# Autodesk Inventor assembly: FLUGGER VALVE ASSY
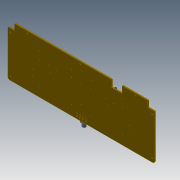
[picture p0: Inventor's stored thumbnail of the model, 180x180]
Saved by Autodesk Inventor 2020.3 (Build 243373000, 373)
## iProperties
RuleStatus: InUse
AfterDocSave0: file://Part Number Cleaner
Created: 2019-10-25
Vendor: HHMI: JRC - ID&F
Document SubType Name: Assembly
Designer: arnoldj
DESIGN DEPARTMENT: HHMI: JRC - ID&F
ALTERED ITEM PART NUMBER: N/A
ALTERED ITEM VENDOR: N/A
ALTERED ITEM DESCRIPTION: N/A
Author: arnoldj
Revision Number: 0
## Documents named in this file (11)
- C:\_WORKSPACE\DATA\PROJECTS\_PROJECTS BY LAB\CARD (LAB)\FLUGGER\FLUGGER VALVE ASSY.iam
- C:\_WORKSPACE\DATA\COMMON\McMaster\MCMASTER 6124K278_AIR DIRECTIONAL CONTROL VALVE.ipt
- C:\_WORKSPACE\DATA\PROJECTS\_PROJECTS BY LAB\CARD (LAB)\FLUGGER\FLUGGER AIR VALVE MTG BRKT.ipt
- C:\_WORKSPACE\DATA\PROJECTS\_PROJECTS BY LAB\CARD (LAB)\FLUGGER\FLUGGER REGULATOR ASSY.iam
- C:\_WORKSPACE\DATA\COMMON\McMaster\MCMASTER 5779K627 WYE.ipt
- C:\_WORKSPACE\DATA\COMMON\McMaster\5779K109_PUSH-TO-CONNECT TUBE FITTING FOR AIR.ipt
- C:\_WORKSPACE\DATA\COMMON\McMaster\MCMASTER 51235K134.ipt
- C:\_WORKSPACE\DATA\COMMON\McMaster\MCMASTER 9164K12.ipt
- C:\_WORKSPACE\DATA\COMMON\Beduan\Beduan 2 WAY NC DC 24V SOLENOID VALVE 0_25 NPT.ipt
- C:\_WORKSPACE\DATA\COMMON\McMaster\MCMASTER 51025K184 PUSH TO CONNECT FITTING.ipt
- C:\_WORKSPACE\DATA\COMMON\McMaster\MCMASTER 5779K36 PUSH TO CONNECT TEE.ipt
## Components (23 placed, 10 different names)
1. FLUGGER AIR VALVE MTG BRKT:1 — Mate:2, Mate:3, Mate:5, Mate:6, Flush:1, Mate:7, Mate:8, Mate:9, Mate:10, Mate:11, Mate:12, Mate:13, Mate:14, Mate:44, Mate:45, Angle:2, Angle:3
2. MCMASTER 6124K278_AIR DIRECTIONAL CONTROL VALVE:1 — Mate:2, Mate:3, Mate:7, Mate:19, Mate:20, Mate:21, Mate:22, Mate:25, Mate:26, Mate:40, Mate:41, Mate:42, Mate:43
3. MCMASTER 6124K278_AIR DIRECTIONAL CONTROL VALVE:2 — Mate:5, Mate:6, Mate:8, Mate:15, Mate:16, Mate:17, Mate:18, Mate:23, Mate:24, Mate:36, Mate:37, Mate:38, Mate:39
4. FLUGGER REGULATOR ASSY:1 [sub-assembly] — Mate:9, Mate:10, Mate:11, Mate:27, Mate:28, Mate:31, Mate:32
5. FLUGGER REGULATOR ASSY:2 [sub-assembly] — Mate:12, Mate:13, Mate:14, Mate:29, Mate:30, Mate:33, Mate:34
6. MCMASTER 5779K627 WYE:1 — Mate:15, Mate:16
7. MCMASTER 5779K627 WYE:2 — Mate:17, Mate:18
8. MCMASTER 5779K627 WYE:3 — Mate:21, Mate:22
9. MCMASTER 5779K627 WYE:4 — Mate:19, Mate:20
10. 5779K109_PUSH-TO-CONNECT TUBE FITTING FOR AIR:1 — Mate:23, Mate:24
11. 5779K109_PUSH-TO-CONNECT TUBE FITTING FOR AIR:2 — Mate:27, Mate:28
12. 5779K109_PUSH-TO-CONNECT TUBE FITTING FOR AIR:3 — Mate:25, Mate:26
13. 5779K109_PUSH-TO-CONNECT TUBE FITTING FOR AIR:4 — Mate:29, Mate:30
14. MCMASTER 51235K134:1 — Mate:31, Mate:32
15. MCMASTER 51235K134:2 — Mate:33, Mate:34, Angle:1
16. MCMASTER 9164K12:1 — Mate:36, Mate:37
17. MCMASTER 9164K12:2 — Mate:38, Mate:39
18. MCMASTER 9164K12:3 — Mate:40, Mate:41
19. MCMASTER 9164K12:4 — Mate:42, Mate:43
20. Beduan 2 WAY NC DC 24V SOLENOID VALVE 0_25 NPT:1 — Mate:44, Mate:45, Angle:2, Mate:46, Mate:47, Mate:48, Mate:49
21. MCMASTER 51025K184 PUSH TO CONNECT FITTING:1 — Mate:46, Mate:47
22. MCMASTER 51025K184 PUSH TO CONNECT FITTING:2 — Mate:48, Mate:49, Mate:50, Mate:51
23. MCMASTER 5779K36 PUSH TO CONNECT TEE:1 — Mate:50, Angle:3, Mate:51
## Relationships (52: Mate 48, Angle 3, Flush 1)
- Mate:2: FLUGGER AIR VALVE MTG BRKT:1 ↔ MCMASTER 6124K278_AIR DIRECTIONAL CONTROL VALVE:1
- Mate:3: FLUGGER AIR VALVE MTG BRKT:1 ↔ MCMASTER 6124K278_AIR DIRECTIONAL CONTROL VALVE:1
- Mate:5: FLUGGER AIR VALVE MTG BRKT:1 ↔ MCMASTER 6124K278_AIR DIRECTIONAL CONTROL VALVE:2
- Mate:6: FLUGGER AIR VALVE MTG BRKT:1 ↔ MCMASTER 6124K278_AIR DIRECTIONAL CONTROL VALVE:2
- Flush:1: FLUGGER AIR VALVE MTG BRKT:1
- Mate:7: FLUGGER AIR VALVE MTG BRKT:1 ↔ MCMASTER 6124K278_AIR DIRECTIONAL CONTROL VALVE:1
- Mate:8: FLUGGER AIR VALVE MTG BRKT:1 ↔ MCMASTER 6124K278_AIR DIRECTIONAL CONTROL VALVE:2
- Mate:9: FLUGGER AIR VALVE MTG BRKT:1 ↔ FLUGGER REGULATOR ASSY:1
- Mate:10: FLUGGER AIR VALVE MTG BRKT:1 ↔ FLUGGER REGULATOR ASSY:1
- Mate:11: FLUGGER AIR VALVE MTG BRKT:1 ↔ FLUGGER REGULATOR ASSY:1
- Mate:12: FLUGGER AIR VALVE MTG BRKT:1 ↔ FLUGGER REGULATOR ASSY:2
- Mate:13: FLUGGER AIR VALVE MTG BRKT:1 ↔ FLUGGER REGULATOR ASSY:2
- Mate:14: FLUGGER AIR VALVE MTG BRKT:1 ↔ FLUGGER REGULATOR ASSY:2
- Mate:15 (2.54 mm): MCMASTER 6124K278_AIR DIRECTIONAL CONTROL VALVE:2 ↔ MCMASTER 5779K627 WYE:1
- Mate:16: MCMASTER 6124K278_AIR DIRECTIONAL CONTROL VALVE:2 ↔ MCMASTER 5779K627 WYE:1
- Mate:17 (2.54 mm): MCMASTER 6124K278_AIR DIRECTIONAL CONTROL VALVE:2 ↔ MCMASTER 5779K627 WYE:2
- Mate:18: MCMASTER 6124K278_AIR DIRECTIONAL CONTROL VALVE:2 ↔ MCMASTER 5779K627 WYE:2
- Mate:19 (2.54 mm): MCMASTER 6124K278_AIR DIRECTIONAL CONTROL VALVE:1 ↔ MCMASTER 5779K627 WYE:4
- Mate:20: MCMASTER 6124K278_AIR DIRECTIONAL CONTROL VALVE:1 ↔ MCMASTER 5779K627 WYE:4
- Mate:21 (2.54 mm): MCMASTER 6124K278_AIR DIRECTIONAL CONTROL VALVE:1 ↔ MCMASTER 5779K627 WYE:3
- Mate:22: MCMASTER 6124K278_AIR DIRECTIONAL CONTROL VALVE:1 ↔ MCMASTER 5779K627 WYE:3
- Mate:23 (2.54 mm): MCMASTER 6124K278_AIR DIRECTIONAL CONTROL VALVE:2 ↔ 5779K109_PUSH-TO-CONNECT TUBE FITTING FOR AIR:1
- Mate:24: MCMASTER 6124K278_AIR DIRECTIONAL CONTROL VALVE:2 ↔ 5779K109_PUSH-TO-CONNECT TUBE FITTING FOR AIR:1
- Mate:25 (2.54 mm): MCMASTER 6124K278_AIR DIRECTIONAL CONTROL VALVE:1 ↔ 5779K109_PUSH-TO-CONNECT TUBE FITTING FOR AIR:3
- Mate:26: MCMASTER 6124K278_AIR DIRECTIONAL CONTROL VALVE:1 ↔ 5779K109_PUSH-TO-CONNECT TUBE FITTING FOR AIR:3
- Mate:27 (2.54 mm): FLUGGER REGULATOR ASSY:1 ↔ 5779K109_PUSH-TO-CONNECT TUBE FITTING FOR AIR:2
- Mate:28: FLUGGER REGULATOR ASSY:1 ↔ 5779K109_PUSH-TO-CONNECT TUBE FITTING FOR AIR:2
- Mate:29 (2.54 mm): FLUGGER REGULATOR ASSY:2 ↔ 5779K109_PUSH-TO-CONNECT TUBE FITTING FOR AIR:4
- Mate:30: FLUGGER REGULATOR ASSY:2 ↔ 5779K109_PUSH-TO-CONNECT TUBE FITTING FOR AIR:4
- Mate:31: FLUGGER REGULATOR ASSY:1 ↔ MCMASTER 51235K134:1
- Mate:32: FLUGGER REGULATOR ASSY:1 ↔ MCMASTER 51235K134:1
- Mate:33: FLUGGER REGULATOR ASSY:2 ↔ MCMASTER 51235K134:2
- Mate:34: FLUGGER REGULATOR ASSY:2 ↔ MCMASTER 51235K134:2
- Angle:1 (180 deg): MCMASTER 51235K134:2
- Mate:36: MCMASTER 6124K278_AIR DIRECTIONAL CONTROL VALVE:2 ↔ MCMASTER 9164K12:1
- Mate:37: MCMASTER 6124K278_AIR DIRECTIONAL CONTROL VALVE:2 ↔ MCMASTER 9164K12:1
- Mate:38: MCMASTER 6124K278_AIR DIRECTIONAL CONTROL VALVE:2 ↔ MCMASTER 9164K12:2
- Mate:39: MCMASTER 6124K278_AIR DIRECTIONAL CONTROL VALVE:2 ↔ MCMASTER 9164K12:2
- Mate:40: MCMASTER 6124K278_AIR DIRECTIONAL CONTROL VALVE:1 ↔ MCMASTER 9164K12:3
- Mate:41: MCMASTER 6124K278_AIR DIRECTIONAL CONTROL VALVE:1 ↔ MCMASTER 9164K12:3
- Mate:42: MCMASTER 6124K278_AIR DIRECTIONAL CONTROL VALVE:1 ↔ MCMASTER 9164K12:4
- Mate:43: MCMASTER 6124K278_AIR DIRECTIONAL CONTROL VALVE:1 ↔ MCMASTER 9164K12:4
- Mate:44: FLUGGER AIR VALVE MTG BRKT:1 ↔ Beduan 2 WAY NC DC 24V SOLENOID VALVE 0_25 NPT:1
- Mate:45: FLUGGER AIR VALVE MTG BRKT:1 ↔ Beduan 2 WAY NC DC 24V SOLENOID VALVE 0_25 NPT:1
- Angle:2 (180 deg): FLUGGER AIR VALVE MTG BRKT:1 ↔ Beduan 2 WAY NC DC 24V SOLENOID VALVE 0_25 NPT:1
- Mate:46: Beduan 2 WAY NC DC 24V SOLENOID VALVE 0_25 NPT:1 ↔ MCMASTER 51025K184 PUSH TO CONNECT FITTING:1
- Mate:47: Beduan 2 WAY NC DC 24V SOLENOID VALVE 0_25 NPT:1 ↔ MCMASTER 51025K184 PUSH TO CONNECT FITTING:1
- Mate:48: Beduan 2 WAY NC DC 24V SOLENOID VALVE 0_25 NPT:1 ↔ MCMASTER 51025K184 PUSH TO CONNECT FITTING:2
- Mate:49: Beduan 2 WAY NC DC 24V SOLENOID VALVE 0_25 NPT:1 ↔ MCMASTER 51025K184 PUSH TO CONNECT FITTING:2
- Mate:50 (12.7 mm): MCMASTER 51025K184 PUSH TO CONNECT FITTING:2 ↔ MCMASTER 5779K36 PUSH TO CONNECT TEE:1
- Angle:3 (0 deg): FLUGGER AIR VALVE MTG BRKT:1 ↔ MCMASTER 5779K36 PUSH TO CONNECT TEE:1
- Mate:51: MCMASTER 51025K184 PUSH TO CONNECT FITTING:2 ↔ MCMASTER 5779K36 PUSH TO CONNECT TEE:1
